# Autodesk Inventor assembly: One simple door
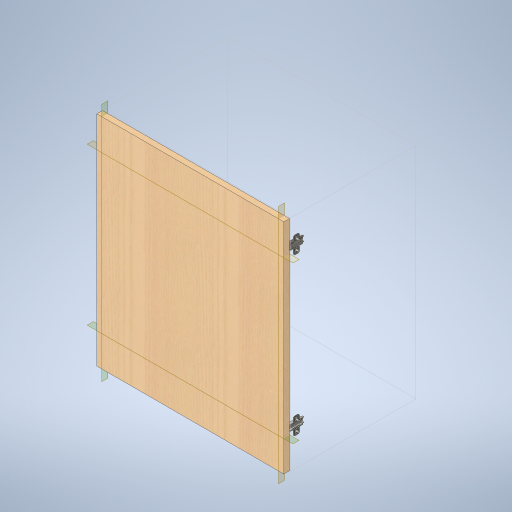
[picture p0: Inventor's stored thumbnail of the model, 512x512]
Saved by Autodesk Inventor 2024 (Build 280153000, 153)
## iProperties
RuleStatus: InUse
Created: 2017-04-11
Part Number: One simple door
Document SubType Name: Assembly
Designer: SvetlanaB
Description: One simple door
Author: SvetlanaB
## Documents named in this file (6)
- C:\W4INV 2024 Design\iBOX LIBRARY\Kitchen\Doors\One simple door\One simple door.iam
- C:\W4INV 2024 Design\iBOX LIBRARY\Kitchen\Doors\One simple door\Door Panel.ipt
- C:\W4INV 2024 Design\iBOX LIBRARY\Kitchen\Doors\One simple door\Simple door Skeleton.ipt
- C:\W4INV 2024 Design\_LIBRARY\Hinges\CONCEALED HINGE\Full Overlay Hinge Wood Screw Cup Wood Screw T18.iam
- C:\W4INV 2023 Design\LIBRARY\Hinges\CONCEALED HINGE.iam
- C:\W4INV 2022 Design\iBOX LIBRARY\Kitchen\Doors\One simple door\One simple door.iam
## Components (4 placed, 3 different names)
1. @Skeleton
2. Door Panel:1 — Flush:1, Flush:2, Flush:3, Flush:4, Mate:5, Mate:7
3. Full Overlay Hinge Wood Screw Cup Wood Screw T18:1 [sub-assembly] — Mate:7, Right bottom hinge, Mate:8, Left bottom hinge
4. Full Overlay Hinge Wood Screw Cup Wood Screw T18:2 [sub-assembly] — Mate:5, Right top hinge, Mate:6, Top left hinge
## Relationships (12: Flush 8, Mate 4)
- Flush:1 (-98.5 mm): Door Panel:1
- Flush:2 (-98.5 mm): Door Panel:1
- Flush:3 (-16.5 mm): Door Panel:1
- Flush:4 (-16.5 mm): Door Panel:1
- Mate:5: Door Panel:1 ↔ Full Overlay Hinge Wood Screw Cup Wood Screw T18:2
- Right top hinge [Flush]: Full Overlay Hinge Wood Screw Cup Wood Screw T18:2
- Mate:6: Full Overlay Hinge Wood Screw Cup Wood Screw T18:2
- Mate:7: Door Panel:1 ↔ Full Overlay Hinge Wood Screw Cup Wood Screw T18:1
- Right bottom hinge [Flush]: Full Overlay Hinge Wood Screw Cup Wood Screw T18:1
- Mate:8: Full Overlay Hinge Wood Screw Cup Wood Screw T18:1
- Top left hinge [Flush]: Full Overlay Hinge Wood Screw Cup Wood Screw T18:2
- Left bottom hinge [Flush]: Full Overlay Hinge Wood Screw Cup Wood Screw T18:1
## Named parameters: Panel_thickness = 18 mm, Left_offset = 1.5 mm, Right_offset = 1.5 mm, Hinge_side_offset = 18 mm, Hinge_top_offset = 100 mm, Hinge_bottom_offset = 100 mm, Width = 600 mm, Depth = 400 mm, Height = 700 mm, Top_offset = 1.5 mm, Bottom_offset = 1.5 mm, Front_offset = 2 mm, Type = 1
